# Autodesk Inventor assembly: Adrian_Cameraarm
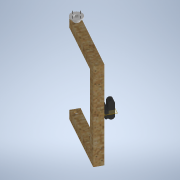
[picture p0: Inventor's stored thumbnail of the model, 180x180]
Saved by Autodesk Inventor 2021 (Build 250183000, 183)
## iProperties
Created: 2022-07-12
Part Number: Adrian_Cameraarm
Document SubType Name: Assembly
Designer: adria
Mass: 1586.11 g
Surface Area: 1802.35 cm^2
Volume: 1534.57 cm^3
Density: 1.03358 g/cm^3
Author: adria
## Documents named in this file (11)
- C:\Users\adria\OneDrive - tum.de\G2_Waste-Recycling\CAD\Adrian_Cameraarm.iam
- C:\Users\adria\OneDrive - tum.de\G2_Waste-Recycling\CAD\Cameralager22.2mitloecher.ipt
- C:\Users\adria\OneDrive - tum.de\G2_Waste-Recycling\CAD\SKF_608.iam
- C:\Users\adria\Documents\Inventor\Content Center Files\R2021\de-DE\ISO 4034(2)\ISO 4034 - M8 - ISO.ipt
- C:\Users\adria\Documents\Inventor\Content Center Files\R2021\de-DE\DIN 125-1  A\DIN 125 - A 8,4.ipt
- C:\Users\adria\Documents\Inventor\Content Center Files\R2021\de-DE\ISO 4762(2)\ISO 4762 - M4 x 16ISO.ipt
- C:\Users\adria\OneDrive - tum.de\G2_Waste-Recycling\CAD\Adrian_Cameraarmseiten.ipt
- C:\Users\adria\Documents\Inventor\Content Center Files\R2021\de-DE\ISO 4762(2)\ISO 4762 - M8 x 50ISO.ipt
- C:\Users\adria\OneDrive - tum.de\G2_Waste-Recycling\CAD\Adrian_Cameraarmoben.ipt
- C:\Users\adria\OneDrive - tum.de\G2_Waste-Recycling\CAD\stepper-motor-nema17-simplified-model-1.snapshot.3\Hikvision_DS-U02.ipt
- C:\Users\adria\OneDrive - tum.de\G2_Waste-Recycling\CAD\Motorcameralager.ipt
## Components (15 placed, 10 different names)
1. Cameralager22.2mitloecher:1 — Passend:11, Passend:12, Passend:13, Passend:14, Passend:24, Fluchtend:1
2. SKF_608:2 [sub-assembly] — Passend:15, Passend:20, Passend:21, Passend:22
3. ISO 4034 M8:1 — Passend:17, Passend:21
4. DIN 125-1 A A 8,4:1 — Passend:15, Passend:20, Passend:23
5. DIN 125-1 A A 8,4:2 — Passend:16, Passend:17
6. Adrian_Cameraarmseiten:1 — Passend:13, Passend:14, Passend:16, Passend:25, Fluchtend:2, Fluchtend:5, Fluchtend:7
7. ISO 4762 M8 x 50:1 — Passend:22, Passend:23, Passend:24, Fluchtend:1
8. Adrian_Cameraarmseiten:2 — Fluchtend:3, Passend:26, Fluchtend:4, Passend:28, Passend:29
9. Adrian_Cameraarmoben:1 — Passend:25, Fluchtend:2, Fluchtend:3, Passend:26, Fluchtend:4, Fluchtend:5, Passend:27, Fluchtend:6
10. Hikvision_DS-U02:1 — Passend:27, Fluchtend:6, Fluchtend:7
11. Motorcameralager:1 — Passend:28, Passend:29
12. ISO 4762 M4 x 16:1 — Passend:11, Passend:12
13. ISO 4762 M4 x 16:2
14. ISO 4762 M4 x 16:3
15. ISO 4762 M4 x 16:4
## Component patterns: (4 elements, first: ISO 4762 M4 x 16:1)
## Relationships (25: Mate 18, Flush 7)
- [Mate]: SKF_608:2 ↔ DIN 125-1 A A 8,4:2
- Passend:11 [Mate]: Cameralager22.2mitloecher:1 ↔ ISO 4762 M4 x 16:1
- Passend:12 [Mate]: Cameralager22.2mitloecher:1 ↔ ISO 4762 M4 x 16:1
- Passend:13 [Mate]: Cameralager22.2mitloecher:1 ↔ Adrian_Cameraarmseiten:1
- Passend:14 [Mate]: Cameralager22.2mitloecher:1 ↔ Adrian_Cameraarmseiten:1
- Passend:15 [Mate]: SKF_608:2 ↔ DIN 125-1 A A 8,4:1
- Passend:16 [Mate]: DIN 125-1 A A 8,4:2 ↔ Adrian_Cameraarmseiten:1
- Passend:17 [Mate]: ISO 4034 M8:1 ↔ DIN 125-1 A A 8,4:2
- Passend:20 [Mate]: SKF_608:2 ↔ DIN 125-1 A A 8,4:1
- Passend:21 [Mate]: SKF_608:2 ↔ ISO 4034 M8:1
- Passend:22 [Mate]: SKF_608:2 ↔ ISO 4762 M8 x 50:1
- Passend:23 [Mate]: DIN 125-1 A A 8,4:1 ↔ ISO 4762 M8 x 50:1
- Passend:24 [Mate]: Cameralager22.2mitloecher:1 ↔ ISO 4762 M8 x 50:1
- Fluchtend:1 [Flush]: Cameralager22.2mitloecher:1 ↔ ISO 4762 M8 x 50:1
- Passend:25 [Mate]: Adrian_Cameraarmseiten:1 ↔ Adrian_Cameraarmoben:1
- Fluchtend:2 [Flush]: Adrian_Cameraarmseiten:1 ↔ Adrian_Cameraarmoben:1
- Fluchtend:3 [Flush]: Adrian_Cameraarmseiten:2 ↔ Adrian_Cameraarmoben:1
- Passend:26 [Mate]: Adrian_Cameraarmseiten:2 ↔ Adrian_Cameraarmoben:1
- Fluchtend:4 [Flush]: Adrian_Cameraarmseiten:2 ↔ Adrian_Cameraarmoben:1
- Fluchtend:5 [Flush]: Adrian_Cameraarmseiten:1 ↔ Adrian_Cameraarmoben:1
- Passend:27 [Mate]: Adrian_Cameraarmoben:1 ↔ Hikvision_DS-U02:1
- Fluchtend:6 [Flush]: Adrian_Cameraarmoben:1 ↔ Hikvision_DS-U02:1
- Fluchtend:7 [Flush] (209.3 mm): Adrian_Cameraarmseiten:1 ↔ Hikvision_DS-U02:1
- Passend:28 [Mate]: Adrian_Cameraarmseiten:2 ↔ Motorcameralager:1
- Passend:29 [Mate]: Adrian_Cameraarmseiten:2 ↔ Motorcameralager:1
